# Autodesk Inventor assembly: Final robot assembly
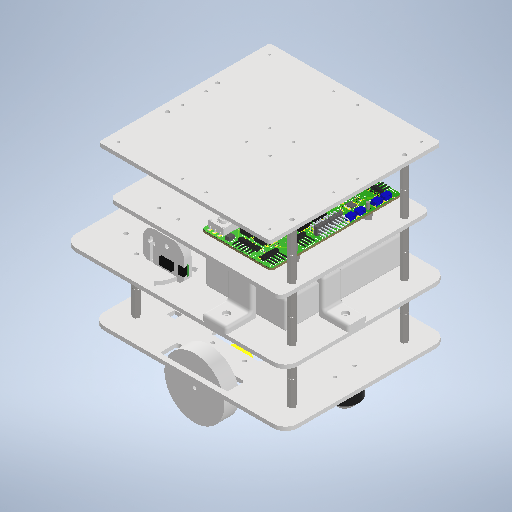
[picture p0: Inventor's stored thumbnail of the model, 512x512]
Saved by Autodesk Inventor 2025.1 (Build 291241000, 241)
## iProperties
Created: 2024-10-04
Part Number: Final robot assembly
Document SubType Name: Assembly
Designer: bw1293
Author: bw1293
## Documents named in this file (9)
- C:\Users\benja\OneDrive\Documents\PlatformIO\Projects\241025-214150-nano33ble\GEOFF-2.0\CAD\Final robot assembly.iam
- C:\Users\benja\OneDrive\Documents\PlatformIO\Projects\241025-214150-nano33ble\GEOFF-2.0\CAD\Bottom layer.iam
- C:\Users\benja\OneDrive\Documents\PlatformIO\Projects\241025-214150-nano33ble\GEOFF-2.0\CAD\Middle layer.iam
- C:\Users\benja\OneDrive\Documents\PlatformIO\Projects\241025-214150-nano33ble\GEOFF-2.0\CAD\Top layer.iam
- C:\Users\benja\OneDrive\Documents\PlatformIO\Projects\241025-214150-nano33ble\GEOFF-2.0\CAD\M2.5 Hex Spacer 20mm 2023.ipt
- C:\Users\benja\OneDrive\Documents\PlatformIO\Projects\241025-214150-nano33ble\GEOFF-2.0\CAD\Battery 2023.ipt
- C:\Users\benja\OneDrive\Documents\PlatformIO\Projects\241025-214150-nano33ble\GEOFF-2.0\CAD\IR Sensor Mount.iam
- C:\Users\benja\OneDrive\Documents\PlatformIO\Projects\241025-214150-nano33ble\GEOFF-2.0\CAD\M2.5 Hex Spacer 20mm.ipt
- C:\Users\benja\OneDrive\Documents\PlatformIO\Projects\241025-214150-nano33ble\GEOFF-2.0\CAD\NeoPixel Base.ipt
## Components (30 placed, 8 different names)
1. Bottom layer:1 [sub-assembly] — Insert:1, Insert:3, Insert:5, Insert:7
2. Middle layer:1 [sub-assembly] — Insert:9, Insert:10, Insert:11, Insert:12, Insert:13, Insert:14, Mate:1, Mate:2, Mate:3
3. IR Sensor Mount:1 [sub-assembly]
4. Top layer:1 [sub-assembly] — Insert:19, Insert:20, Insert:21, Insert:22, Insert:25, Insert:27
5. M2.5 Hex Spacer 20mm 2023:1 — Insert:3, Insert:4
6. M2.5 Hex Spacer 20mm 2023:2 — Insert:1, Insert:2
7. M2.5 Hex Spacer 20mm 2023:3 — Insert:5, Insert:6
8. M2.5 Hex Spacer 20mm 2023:4 — Insert:2
9. M2.5 Hex Spacer 20mm 2023:5 — Insert:7, Insert:8
10. M2.5 Hex Spacer 20mm 2023:6 — Insert:4, Insert:10
11. M2.5 Hex Spacer 20mm 2023:7 — Insert:8
12. M2.5 Hex Spacer 20mm 2023:8 — Insert:6, Insert:9
13. M2.5 Hex Spacer 20mm 2023:9 — Insert:15, Insert:20
14. M2.5 Hex Spacer 20mm 2023:10 — Insert:16
15. M2.5 Hex Spacer 20mm 2023:11 — Insert:17
16. M2.5 Hex Spacer 20mm 2023:12 — Insert:18, Insert:19
17. M2.5 Hex Spacer 20mm 2023:13 — Insert:13, Insert:17
18. M2.5 Hex Spacer 20mm 2023:14 — Insert:14, Insert:18
19. M2.5 Hex Spacer 20mm 2023:15 — Insert:12, Insert:16
20. M2.5 Hex Spacer 20mm 2023:16 — Insert:11, Insert:15
21. Battery 2023:1 — Mate:1, Mate:2, Mate:3
22. M2.5 Hex Spacer 20mm:1 — Insert:21, Insert:23
23. M2.5 Hex Spacer 20mm:2 — Insert:22, Insert:24
24. M2.5 Hex Spacer 20mm:3 — Insert:24, Insert:29
25. M2.5 Hex Spacer 20mm:4 — Insert:25, Insert:26
26. M2.5 Hex Spacer 20mm:5 — Insert:23
27. M2.5 Hex Spacer 20mm:6 — Insert:28, Insert:30
28. M2.5 Hex Spacer 20mm:7 — Insert:27, Insert:28
29. M2.5 Hex Spacer 20mm:8 — Insert:26
30. NeoPixel Base:1 — Insert:29, Insert:30
## Relationships (33: Insert 30, Mate 3)
- Insert:1: Bottom layer:1 ↔ M2.5 Hex Spacer 20mm 2023:2
- Insert:2: M2.5 Hex Spacer 20mm 2023:2 ↔ M2.5 Hex Spacer 20mm 2023:4
- Insert:3: Bottom layer:1 ↔ M2.5 Hex Spacer 20mm 2023:1
- Insert:4: M2.5 Hex Spacer 20mm 2023:1 ↔ M2.5 Hex Spacer 20mm 2023:6
- Insert:5: Bottom layer:1 ↔ M2.5 Hex Spacer 20mm 2023:3
- Insert:6: M2.5 Hex Spacer 20mm 2023:3 ↔ M2.5 Hex Spacer 20mm 2023:8
- Insert:7: Bottom layer:1 ↔ M2.5 Hex Spacer 20mm 2023:5
- Insert:8: M2.5 Hex Spacer 20mm 2023:5 ↔ M2.5 Hex Spacer 20mm 2023:7
- Insert:9: Middle layer:1 ↔ M2.5 Hex Spacer 20mm 2023:8
- Insert:10: Middle layer:1 ↔ M2.5 Hex Spacer 20mm 2023:6
- Insert:11: Middle layer:1 ↔ M2.5 Hex Spacer 20mm 2023:16
- Insert:12: Middle layer:1 ↔ M2.5 Hex Spacer 20mm 2023:15
- Insert:13: Middle layer:1 ↔ M2.5 Hex Spacer 20mm 2023:13
- Insert:14: Middle layer:1 ↔ M2.5 Hex Spacer 20mm 2023:14
- Insert:15: M2.5 Hex Spacer 20mm 2023:9 ↔ M2.5 Hex Spacer 20mm 2023:16
- Insert:16: M2.5 Hex Spacer 20mm 2023:10 ↔ M2.5 Hex Spacer 20mm 2023:15
- Insert:17: M2.5 Hex Spacer 20mm 2023:11 ↔ M2.5 Hex Spacer 20mm 2023:13
- Insert:18: M2.5 Hex Spacer 20mm 2023:12 ↔ M2.5 Hex Spacer 20mm 2023:14
- Mate:1: Middle layer:1 ↔ Battery 2023:1
- Mate:2: Middle layer:1 ↔ Battery 2023:1
- Mate:3: Middle layer:1 ↔ Battery 2023:1
- Insert:19: Top layer:1 ↔ M2.5 Hex Spacer 20mm 2023:12
- Insert:20: Top layer:1 ↔ M2.5 Hex Spacer 20mm 2023:9
- Insert:21: Top layer:1 ↔ M2.5 Hex Spacer 20mm:1
- Insert:22: Top layer:1 ↔ M2.5 Hex Spacer 20mm:2
- Insert:23: M2.5 Hex Spacer 20mm:1 ↔ M2.5 Hex Spacer 20mm:5
- Insert:24: M2.5 Hex Spacer 20mm:2 ↔ M2.5 Hex Spacer 20mm:3
- Insert:25: Top layer:1 ↔ M2.5 Hex Spacer 20mm:4
- Insert:26: M2.5 Hex Spacer 20mm:4 ↔ M2.5 Hex Spacer 20mm:8
- Insert:27: Top layer:1 ↔ M2.5 Hex Spacer 20mm:7
- Insert:28: M2.5 Hex Spacer 20mm:6 ↔ M2.5 Hex Spacer 20mm:7
- Insert:29: M2.5 Hex Spacer 20mm:3 ↔ NeoPixel Base:1
- Insert:30: M2.5 Hex Spacer 20mm:6 ↔ NeoPixel Base:1
